# Autodesk Inventor assembly: Assembly5
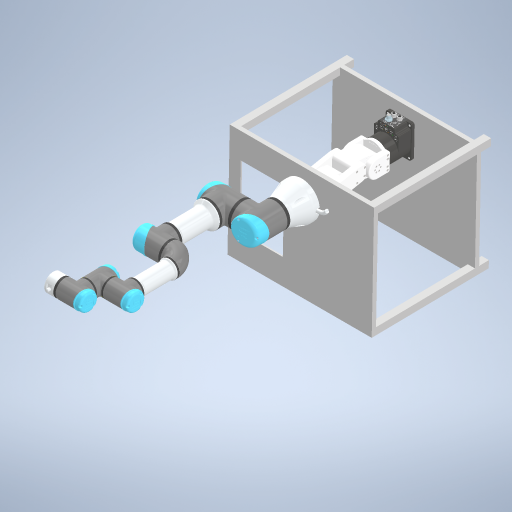
[picture p0: Inventor's stored thumbnail of the model, 512x512]
Saved by Autodesk Inventor 2023 (Build 270158000, 158)
## iProperties
Created: 2022-09-30
Part Number: Assembly5
Document SubType Name: Assembly
Designer: benni
Author: benni
## Documents named in this file (4)
- C:\Users\benni\Documents\Studium\7. Semester\Industrial Robotics\Assignment 2\@Table\Assembly5.iam
- C:\Users\benni\Downloads\ur3step\UR3.iam
- C:\Users\benni\Documents\Studium\7. Semester\Industrial Robotics\Assignment 2\@Table\Table.ipt
- C:\Users\benni\Downloads\meca500-robot-assembled-stp\Meca500 Assembly simple.iam
## Components (3 placed, 3 different names)
1. UR3:1 [sub-assembly] — Mate:1, Mate:2, Flush:1
2. Table:1 — Mate:1, Mate:2, Flush:1, Mate:3, Flush:2, Mate:4
3. Meca500 Assembly simple:1 [sub-assembly] — Mate:3, Flush:2, Mate:4
## Relationships (6: Mate 4, Flush 2)
- Mate:1: UR3:1 ↔ Table:1
- Mate:2: UR3:1 ↔ Table:1
- Flush:1 (101.6 mm): UR3:1 ↔ Table:1
- Mate:3: Table:1 ↔ Meca500 Assembly simple:1
- Flush:2 (820 mm): Table:1 ↔ Meca500 Assembly simple:1
- Mate:4 (330 mm): Table:1 ↔ Meca500 Assembly simple:1
